# Autodesk Inventor assembly: Сборка3
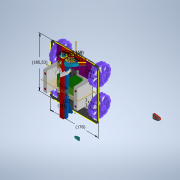
[picture p0: Inventor's stored thumbnail of the model, 180x180]
Saved by Autodesk Inventor 2020 (Build 240168000, 168)
## iProperties
Created: 2022-07-29
Part Number: Сборка3
Document SubType Name: Assembly
Designer: akapu
Author: akapu
## Documents named in this file (25)
- C:\Users\akapu\Documents\maze bot\Сборка3.iam
- C:\Users\akapu\Documents\maze bot\maze_04.ipt
- C:\Users\akapu\Documents\maze bot\motor.ipt
- C:\Users\akapu\Documents\maze bot\motor_ЗЕРКАЛО.ipt
- C:\Users\akapu\Documents\maze bot\akkum_holder_up.ipt
- C:\Users\akapu\Documents\maze bot\akkum_holder.ipt
- C:\Users\akapu\Documents\maze bot\metal_holder.ipt
- C:\Users\akapu\Documents\maze bot\rama.ipt
- C:\Users\akapu\Documents\maze bot\vydacha_4.ipt
- C:\Users\akapu\Documents\maze bot\pizza.ipt
- C:\Users\akapu\Documents\maze bot\pizza_disk.ipt
- C:\Users\akapu\Documents\maze bot\pizza_2.ipt
- C:\Users\akapu\Documents\maze bot\mg996r v17.iam
- C:\Users\akapu\Documents\maze bot\reyka_3.ipt
- C:\Users\akapu\Documents\maze bot\lid.ipt
- C:\Users\akapu\Documents\maze bot\vagonetka_2.ipt
- C:\Users\akapu\Documents\maze bot\wheel_5.ipt
- C:\Users\akapu\Documents\maze bot\block.ipt
- C:\Users\akapu\Documents\maze bot\rolik_2.ipt
- C:\Users\akapu\Documents\maze bot\защёлка_выдача2.ipt
- C:\Users\akapu\Documents\maze bot\держатель_гаек.ipt
- C:\Users\akapu\Documents\maze bot\разделитель.ipt
- C:\Users\akapu\Documents\maze bot\block_01.ipt
- C:\Users\akapu\Documents\maze bot\block_02.ipt
- C:\Users\akapu\Documents\maze bot\Деталь2.ipt
## Components (32 placed, 24 different names)
1. maze_04:1 — С поворотом:1, С поворотом:2, С поворотом:3, С поворотом:4, Вставка:1, Вставка:2, Вставка:4, С поворотом:5, Совмещение:7, Совмещение:8, Совмещение:9, Совмещение:11, Совмещение:12, Совмещение:13, Совмещение:17, Совмещение:27, Совмещение:31, Совмещение:32, Совмещение:33, Совмещение:34, Совмещение:35, Совмещение:36, Совмещение:37, Заподлицо:1, Заподлицо:2, Совмещение:51
2. motor:1 — С поворотом:1, Совмещение:12, Вставка:6, Совмещение:29
3. motor:2 — С поворотом:2, Совмещение:8, Вставка:8, Совмещение:28
4. motor_ЗЕРКАЛО:1 — С поворотом:3, Совмещение:7, Вставка:7, Совмещение:26
5. motor_ЗЕРКАЛО:2 — С поворотом:4, Совмещение:9, Совмещение:10, Совмещение:11, Вставка:9, Совмещение:30
6. akkum_holder_up:1 — Вставка:1, Совмещение:13
7. akkum_holder:1 — Вставка:2, Вставка:3
8. metal_holder:1 — Вставка:3, Совмещение:17
9. rama:1 — Вставка:4, С поворотом:5, С поворотом:6, С поворотом:7, Совмещение:18, Совмещение:48
10. vydacha_4:1 — С поворотом:6, Совмещение:10, Совмещение:45, Совмещение:46, Совмещение:47
11. pizza:1 — С поворотом:7, Совмещение:2, Совмещение:3, Совмещение:18, С поворотом:8, Совмещение:19, Угол:2, Совмещение:49
12. pizza_disk:1 — Совмещение:2, Совмещение:3, Угол:2
13. pizza_2:1 — Совмещение:48, Совмещение:49
14. mg996r v17:1 [sub-assembly] — Совмещение:45, Совмещение:46, Совмещение:47
15. reyka_3:1 — С поворотом:8, Совмещение:19, Вставка:5, Совмещение:20, Совмещение:21, Угол:1, Совмещение:42
16. lid:1 — Вставка:5, Совмещение:23, Совмещение:24, Совмещение:25, Совмещение:39, Совмещение:40, Совмещение:41, Угол:1, Совмещение:43, Совмещение:50
17. vagonetka_2:1 — Совмещение:20, Совмещение:21, Совмещение:42
18. wheel_5:1 — Вставка:6
19. wheel_5:2 — Вставка:7
20. wheel_5:3 — Вставка:9
21. wheel_5:4 — Вставка:8
22. block:1
23. rolik_2:1 — Совмещение:43, Совмещение:50
24. защёлка_выдача2:1 — Совмещение:23, Совмещение:24, Совмещение:25
25. держатель_гаек:1 — Совмещение:26, Совмещение:27, Совмещение:35
26. держатель_гаек:2 — Совмещение:28, Совмещение:32, Совмещение:34
27. держатель_гаек:3 — Совмещение:29, Совмещение:33, Совмещение:36
28. держатель_гаек:4 — Совмещение:30, Совмещение:31, Совмещение:37
29. разделитель:1 — Совмещение:39, Совмещение:40, Совмещение:41
30. block_01:1 — Вставка:11
31. block_02:1 — Вставка:11
32. Деталь2:1 — Заподлицо:1, Заподлицо:2, Совмещение:51
## Relationships (63: Mate 41, Insert 10, RevoluteJoint 8, Angle 2, Flush 2)
- С поворотом:1 [RevoluteJoint]: maze_04:1 ↔ motor:1
- С поворотом:2 [RevoluteJoint]: maze_04:1 ↔ motor:2
- С поворотом:3 [RevoluteJoint]: maze_04:1 ↔ motor_ЗЕРКАЛО:1
- С поворотом:4 [RevoluteJoint]: maze_04:1 ↔ motor_ЗЕРКАЛО:2
- Вставка:1 [Insert]: maze_04:1 ↔ akkum_holder_up:1
- Вставка:2 [Insert]: maze_04:1 ↔ akkum_holder:1
- Вставка:3 [Insert]: akkum_holder:1 ↔ metal_holder:1
- Вставка:4 [Insert]: maze_04:1 ↔ rama:1
- С поворотом:5 [RevoluteJoint]: maze_04:1 ↔ rama:1
- С поворотом:6 [RevoluteJoint]: rama:1 ↔ vydacha_4:1
- С поворотом:7 [RevoluteJoint]: rama:1 ↔ pizza:1
- Совмещение:2 [Mate]: pizza:1 ↔ pizza_disk:1
- Совмещение:3 [Mate]: pizza:1 ↔ pizza_disk:1
- Совмещение:7 [Mate]: maze_04:1 ↔ motor_ЗЕРКАЛО:1
- Совмещение:8 [Mate]: maze_04:1 ↔ motor:2
- Совмещение:9 [Mate]: maze_04:1 ↔ motor_ЗЕРКАЛО:2
- Совмещение:10 [Mate]: motor_ЗЕРКАЛО:2 ↔ vydacha_4:1
- Совмещение:11 [Mate]: maze_04:1 ↔ motor_ЗЕРКАЛО:2
- Совмещение:12 [Mate]: maze_04:1 ↔ motor:1
- Совмещение:13 [Mate]: maze_04:1 ↔ akkum_holder_up:1
- Совмещение:17 [Mate]: maze_04:1 ↔ metal_holder:1
- Совмещение:18 [Mate]: rama:1 ↔ pizza:1
- С поворотом:8 [RevoluteJoint]: pizza:1 ↔ reyka_3:1
- Совмещение:19 [Mate]: pizza:1 ↔ reyka_3:1
- Вставка:5 [Insert] (0.5 mm): reyka_3:1 ↔ lid:1
- Совмещение:20 [Mate]: reyka_3:1 ↔ vagonetka_2:1
- Совмещение:21 [Mate]: reyka_3:1 ↔ vagonetka_2:1
- Вставка:6 [Insert]: motor:1 ↔ wheel_5:1
- Вставка:7 [Insert]: motor_ЗЕРКАЛО:1 ↔ wheel_5:2
- Вставка:8 [Insert]: motor:2 ↔ wheel_5:4
- Вставка:9 [Insert]: motor_ЗЕРКАЛО:2 ↔ wheel_5:3
- Совмещение:23 [Mate]: lid:1 ↔ защёлка_выдача2:1
- Совмещение:24 [Mate] (-5.2 mm): lid:1 ↔ защёлка_выдача2:1
- Совмещение:25 [Mate]: lid:1 ↔ защёлка_выдача2:1
- Совмещение:26 [Mate]: motor_ЗЕРКАЛО:1 ↔ держатель_гаек:1
- Совмещение:27 [Mate]: maze_04:1 ↔ держатель_гаек:1
- Совмещение:28 [Mate]: motor:2 ↔ держатель_гаек:2
- Совмещение:29 [Mate]: motor:1 ↔ держатель_гаек:3
- Совмещение:30 [Mate]: motor_ЗЕРКАЛО:2 ↔ держатель_гаек:4
- Совмещение:31 [Mate]: maze_04:1 ↔ держатель_гаек:4
- Совмещение:32 [Mate]: maze_04:1 ↔ держатель_гаек:2
- Совмещение:33 [Mate]: maze_04:1 ↔ держатель_гаек:3
- Совмещение:34 [Mate]: maze_04:1 ↔ держатель_гаек:2
- Совмещение:35 [Mate]: maze_04:1 ↔ держатель_гаек:1
- Совмещение:36 [Mate]: maze_04:1 ↔ держатель_гаек:3
- Совмещение:37 [Mate]: maze_04:1 ↔ держатель_гаек:4
- Совмещение:39 [Mate]: lid:1 ↔ разделитель:1
- Совмещение:40 [Mate]: lid:1 ↔ разделитель:1
- Совмещение:41 [Mate]: lid:1 ↔ разделитель:1
- Угол:1 [Angle] (0 deg): reyka_3:1 ↔ lid:1
- Угол:2 [Angle] (0 deg): pizza:1 ↔ pizza_disk:1
- Совмещение:42 [Mate]: reyka_3:1 ↔ vagonetka_2:1
- Вставка:11 [Insert] (-3 mm): block_01:1 ↔ block_02:1
- Совмещение:43 [Mate]: lid:1 ↔ rolik_2:1
- Совмещение:45 [Mate]: vydacha_4:1 ↔ mg996r v17:1
- Совмещение:46 [Mate]: vydacha_4:1 ↔ mg996r v17:1
- Совмещение:47 [Mate]: vydacha_4:1 ↔ mg996r v17:1
- Совмещение:48 [Mate] (-3 mm): rama:1 ↔ pizza_2:1
- Совмещение:49 [Mate]: pizza:1 ↔ pizza_2:1
- Совмещение:50 [Mate]: lid:1 ↔ rolik_2:1
- Заподлицо:1 [Flush]: maze_04:1 ↔ Деталь2:1
- Заподлицо:2 [Flush]: maze_04:1 ↔ Деталь2:1
- Совмещение:51 [Mate]: maze_04:1 ↔ Деталь2:1
